# Autodesk Inventor assembly: Table_Setup_2
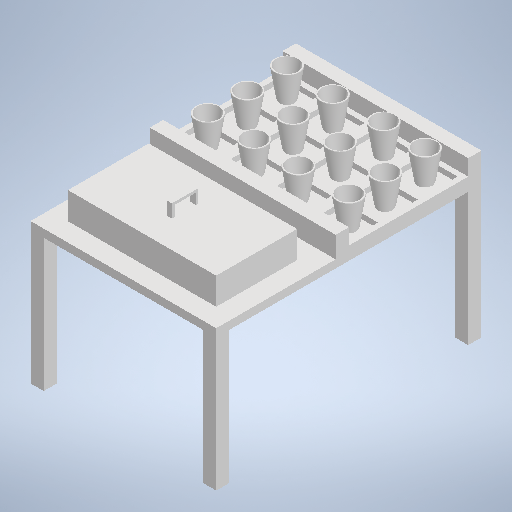
[picture p0: Inventor's stored thumbnail of the model, 512x512]
Saved by Autodesk Inventor 2025 (Build 290162000, 162)
## iProperties
Created: 2024-07-31
Part Number: Table_Setup_2
Document SubType Name: Assembly
Designer: User
Author: User
## Documents named in this file (4)
- C:\Users\User\OneDrive\Documents\FYP\Inventor_Designs\Setups\Table_Setup_2.iam
- C:\Users\User\OneDrive\Documents\FYP\Inventor_Designs\Platform\Table_2.ipt
- C:\Users\User\OneDrive\Documents\FYP\Inventor_Designs\Platform\Blackout Box.ipt
- C:\Users\User\OneDrive\Documents\FYP\Inventor_Designs\Rack\Cup for seeds.ipt
## Components (14 placed, 3 different names)
1. Table_2:1 — Mate:1, Flush:1, Flush:2, Mate:2, Mate:3, Mate:5, Mate:6, Mate:7, Mate:9, Mate:11, Mate:12, Mate:13, Mate:14, Mate:15, Mate:16
2. Blackout Box:3 — Mate:1, Flush:1, Flush:2
3. Cup for seeds:1 — Mate:2
4. Cup for seeds:2 — Mate:3
5. Cup for seeds:3 — Mate:7
6. Cup for seeds:4 — Mate:6
7. Cup for seeds:7 — Mate:11
8. Cup for seeds:8 — Mate:12
9. Cup for seeds:9 — Mate:13
10. Cup for seeds:10 — Mate:14
11. Cup for seeds:12 — Mate:15
12. Cup for seeds:13 — Mate:16
13. Cup for seeds:19 — Mate:9
14. Cup for seeds:20 — Mate:5
## Relationships (15: Mate 13, Flush 2)
- Mate:1: Table_2:1 ↔ Blackout Box:3
- Flush:1 (70 mm): Table_2:1 ↔ Blackout Box:3
- Flush:2 (70 mm): Table_2:1 ↔ Blackout Box:3
- Mate:2: Table_2:1 ↔ Cup for seeds:1
- Mate:3: Table_2:1 ↔ Cup for seeds:2
- Mate:5: Table_2:1 ↔ Cup for seeds:20
- Mate:6: Table_2:1 ↔ Cup for seeds:4
- Mate:7: Table_2:1 ↔ Cup for seeds:3
- Mate:9: Table_2:1 ↔ Cup for seeds:19
- Mate:11: Table_2:1 ↔ Cup for seeds:7
- Mate:12: Table_2:1 ↔ Cup for seeds:8
- Mate:13: Table_2:1 ↔ Cup for seeds:9
- Mate:14: Table_2:1 ↔ Cup for seeds:10
- Mate:15: Table_2:1 ↔ Cup for seeds:12
- Mate:16: Table_2:1 ↔ Cup for seeds:13
